# Autodesk Inventor assembly: Quadcopter Assembly
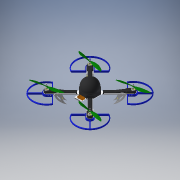
[picture p0: Inventor's stored thumbnail of the model, 180x180]
Saved by Autodesk Inventor 2016 (Build 200138000, 138)
## iProperties
Created: 2015-05-14
Part Number: Quadcopter Assembly
Document SubType Name: Assembly
Designer: Admin
Author: Admin
## Documents named in this file (16)
- E:\Documents\GITHUB\Side-Projects\Quadcopter\Quadcopter Assembly.iam
- E:\Documents\GITHUB\Side-Projects\Quadcopter\Arm.ipt
- E:\Documents\GITHUB\Side-Projects\Quadcopter\Body.ipt
- E:\Documents\GITHUB\Side-Projects\Quadcopter\ArmCover.ipt
- E:\Documents\GITHUB\Side-Projects\Quadcopter\MotorFull.ipt
- E:\Documents\GITHUB\Side-Projects\Quadcopter\Drone propeller guard.ipt
- E:\Documents\GITHUB\Side-Projects\Quadcopter\Motor top.ipt
- E:\Documents\GITHUB\Side-Projects\Quadcopter\propeller.ipt
- E:\Documents\GITHUB\Side-Projects\Quadcopter\Drone Cover.ipt
- E:\Documents\GITHUB\Side-Projects\Quadcopter\landing-gear-ublock.ipt
- E:\Documents\GITHUB\Side-Projects\Quadcopter\landing-gear-claws.ipt
- E:\Documents\GITHUB\Side-Projects\Quadcopter\clawholder.ipt
- E:\Documents\GITHUB\Side-Projects\Quadcopter\screw.ipt
- E:\Documents\GITHUB\Side-Projects\Quadcopter\control board.ipt
- E:\Documents\GITHUB\Side-Projects\Quadcopter\receiver.ipt
- E:\Documents\GITHUB\Side-Projects\Quadcopter\nut.ipt
## Components (112 placed, 15 different names)
1. Arm:1 — Mate:3, Rotational:2, Mate:8, Mate:32, Mate:35, Mate:52
2. Arm:2 — Mate:4, Rotational:4, Mate:10, Mate:17, Mate:18, Mate:28, Mate:29
3. Arm:3 — Mate:2, Rotational:3, Mate:5, Mate:13, Mate:14, Mate:49, Mate:50
4. Arm:4 — Mate:1, Rotational:1, Mate:12, Mate:43, Mate:44, Mate:45, Mate:46, Mate:47
5. Body:1 — Rotational:1, Rotational:2, Rotational:3, Rotational:4, Mate:25, Mate:26, Mate:27, Mate:51, Insert:5, Insert:6, Insert:7, Insert:8, Insert:9, Insert:10, Insert:11, Insert:12, Mate:53, Mate:54
6. ArmCover:1 — Mate:8
7. ArmCover:2 — Mate:5
8. ArmCover:3 — Mate:12
9. ArmCover:4 — Mate:10
10. MotorFull:1 — Mate:4, Mate:21
11. MotorFull:2 — Mate:3, Mate:24
12. MotorFull:3 — Mate:2, Mate:23
13. MotorFull:4 — Mate:1, Mate:22
14. Drone propeller guard:1 — Mate:13, Mate:14, Insert:49, Insert:50, Insert:59, Insert:60
15. Drone propeller guard:2 — Mate:52, Insert:55, Insert:56, Insert:61, Insert:62
16. Drone propeller guard:3 — Mate:17, Mate:18, Insert:53, Insert:54, Insert:63, Insert:64
17. Drone propeller guard:4 — Mate:43, Mate:44, Mate:45, Insert:51, Insert:52, Insert:57, Insert:58
18. Motor top:1 — Mate:24, Rotational:6, Insert:16, Insert:17, Insert:18
19. Motor top:2 — Mate:23, Rotational:8, Insert:13, Insert:14, Insert:15
20. Motor top:3 — Mate:22, Rotational:5, Insert:22, Insert:23, Insert:24
21. Motor top:4 — Mate:21, Rotational:7, Insert:19, Insert:20, Insert:21
22. propeller:1 — Rotational:5, Mate:58
23. propeller:2 — Rotational:6, Mate:55
24. propeller:3 — Rotational:7, Mate:57
25. propeller:4 — Rotational:8, Mate:56
26. Drone Cover:1 — Mate:25, Mate:26, Mate:27
27. landing-gear-ublock:2 — Mate:32, Mate:35, Rotational:9, Rotational:12
28. landing-gear-ublock:4 — Mate:28, Mate:29, Rotational:13, Rotational:15
29. landing-gear-claws:2 — Rotational:12, Mate:37, Insert:25, Insert:26, Insert:27
30. landing-gear-claws:3 — Rotational:13, Mate:41, Insert:31, Insert:32, Insert:48
31. landing-gear-claws:4 — Rotational:15, Mate:40, Insert:36, Insert:37, Insert:38
32. landing-gear-claws:5 — Mate:38, Rotational:17, Insert:28, Insert:29, Insert:30
33. landing-gear-claws:6 — Rotational:16, Mate:48, Insert:42, Insert:43, Insert:44
34. landing-gear-claws:7 — Rotational:9, Mate:36, Insert:39, Insert:40, Insert:41
35. clawholder:1
36. clawholder:2 — Mate:40, Mate:41
37. clawholder:3 — Mate:36, Mate:37
38. clawholder:4 — Mate:38, Mate:48
39. landing-gear-ublock:5 — Mate:46, Mate:47, Rotational:16, Rotational:17
40. landing-gear-ublock:6 — Mate:49, Mate:50, Rotational:18, Rotational:19
41. landing-gear-claws:8 — Rotational:18, Insert:45, Insert:46, Insert:47
42. landing-gear-claws:9 — Rotational:19, Insert:33, Insert:34, Insert:35
43. screw:1 — Insert:59
44. screw:2 — Insert:48
45. screw:3 — Insert:55
46. screw:4 — Insert:47
47. screw:5 — Insert:37
48. screw:6 — Insert:43
49. screw:7 — Insert:36
50. screw:8 — Insert:23
51. screw:9 — Insert:57
52. screw:10 — Insert:64
53. screw:11 — Insert:49
54. screw:12 — Insert:21
55. screw:13 — Insert:15
56. screw:14 — Insert:14
57. screw:15 — Insert:56
58. screw:19 — Insert:13
59. screw:20 — Insert:52
60. screw:21 — Insert:60
61. screw:22 — Insert:35
62. screw:23 — Insert:46
63. screw:24 — Insert:51
64. screw:25 — Insert:50
65. screw:26 — Insert:30
66. screw:27 — Insert:26
67. screw:28 — Insert:1
68. screw:29 — Insert:2
69. screw:30 — Insert:6
70. screw:31 — Insert:4
71. screw:32 — Insert:5
72. screw:33 — Insert:7
73. screw:34 — Insert:3
74. screw:35 — Insert:10
75. screw:36 — Insert:18
76. screw:37 — Insert:33
77. screw:38 — Insert:31
78. screw:39 — Insert:38
79. screw:40 — Insert:41
80. screw:41 — Insert:39
81. screw:43 — Insert:63
82. screw:44 — Insert:62
83. screw:45 — Insert:61
84. screw:46 — Insert:54
85. screw:47 — Insert:42
86. screw:48 — Insert:44
87. screw:49 — Insert:34
88. screw:50 — Insert:27
89. screw:51 — Insert:16
90. screw:52 — Insert:11
91. screw:53 — Insert:9
92. screw:54 — Insert:8
93. screw:55 — Insert:12
94. screw:56 — Insert:25
95. screw:57 — Insert:19
96. screw:58 — Insert:53
97. screw:59 — Insert:40
98. screw:60 — Insert:58
99. screw:61 — Insert:32
100. screw:62 — Insert:22
101. screw:63 — Insert:20
102. screw:64 — Insert:45
103. screw:65 — Insert:29
104. screw:66 — Insert:28
105. screw:67 — Insert:17
106. screw:68 — Insert:24
107. control board:1 — Mate:51, Insert:1, Insert:2, Insert:3, Insert:4
108. receiver:1 — Mate:53, Mate:54
109. nut:1 — Mate:57
110. nut:2 — Mate:55
111. nut:3 — Mate:58
112. nut:4 — Mate:56
## Relationships (124: Insert 64, Mate 44, RevoluteJoint 16)
- Mate:1: Arm:4 ↔ MotorFull:4
- Mate:2: Arm:3 ↔ MotorFull:3
- Mate:3: Arm:1 ↔ MotorFull:2
- Mate:4: Arm:2 ↔ MotorFull:1
- Rotational:1 [RevoluteJoint]: Arm:4 ↔ Body:1
- Rotational:2 [RevoluteJoint]: Arm:1 ↔ Body:1
- Rotational:3 [RevoluteJoint]: Arm:3 ↔ Body:1
- Rotational:4 [RevoluteJoint]: Arm:2 ↔ Body:1
- Mate:5: Arm:3 ↔ ArmCover:2
- Mate:8: Arm:1 ↔ ArmCover:1
- Mate:10: Arm:2 ↔ ArmCover:4
- Mate:12: Arm:4 ↔ ArmCover:3
- Mate:13: Arm:3 ↔ Drone propeller guard:1
- Mate:14: Arm:3 ↔ Drone propeller guard:1
- Mate:17: Arm:2 ↔ Drone propeller guard:3
- Mate:18: Arm:2 ↔ Drone propeller guard:3
- Mate:21: MotorFull:1 ↔ Motor top:4
- Mate:22: MotorFull:4 ↔ Motor top:3
- Mate:23: MotorFull:3 ↔ Motor top:2
- Mate:24: MotorFull:2 ↔ Motor top:1
- Rotational:5 [RevoluteJoint] (-4.5974 mm): Motor top:3 ↔ propeller:1
- Rotational:6 [RevoluteJoint] (-4.5974 mm): Motor top:1 ↔ propeller:2
- Rotational:7 [RevoluteJoint] (4.5974 mm): Motor top:4 ↔ propeller:3
- Rotational:8 [RevoluteJoint] (-4.5974 mm): Motor top:2 ↔ propeller:4
- Mate:25: Body:1 ↔ Drone Cover:1
- Mate:26: Body:1 ↔ Drone Cover:1
- Mate:27: Body:1 ↔ Drone Cover:1
- Mate:28: Arm:2 ↔ landing-gear-ublock:4
- Mate:29: Arm:2 ↔ landing-gear-ublock:4
- Mate:32: Arm:1 ↔ landing-gear-ublock:2
- Mate:35: Arm:1 ↔ landing-gear-ublock:2
- Rotational:9 [RevoluteJoint]: landing-gear-ublock:2 ↔ landing-gear-claws:7
- Rotational:12 [RevoluteJoint]: landing-gear-ublock:2 ↔ landing-gear-claws:2
- Rotational:13 [RevoluteJoint]: landing-gear-ublock:4 ↔ landing-gear-claws:3
- Rotational:15 [RevoluteJoint]: landing-gear-ublock:4 ↔ landing-gear-claws:4
- Mate:36: landing-gear-claws:7 ↔ clawholder:3
- Mate:37: landing-gear-claws:2 ↔ clawholder:3
- Mate:38: landing-gear-claws:5 ↔ clawholder:4
- Mate:40: landing-gear-claws:4 ↔ clawholder:2
- Mate:41: landing-gear-claws:3 ↔ clawholder:2
- Mate:43: Arm:4 ↔ Drone propeller guard:4
- Mate:44: Arm:4 ↔ Drone propeller guard:4
- Mate:45: Arm:4 ↔ Drone propeller guard:4
- Mate:46: Arm:4 ↔ landing-gear-ublock:5
- Mate:47: Arm:4 ↔ landing-gear-ublock:5
- Rotational:16 [RevoluteJoint]: landing-gear-claws:6 ↔ landing-gear-ublock:5
- Rotational:17 [RevoluteJoint]: landing-gear-claws:5 ↔ landing-gear-ublock:5
- Mate:48: landing-gear-claws:6 ↔ clawholder:4
- Mate:49: Arm:3 ↔ landing-gear-ublock:6
- Mate:50: Arm:3 ↔ landing-gear-ublock:6
- Rotational:18 [RevoluteJoint]: landing-gear-ublock:6 ↔ landing-gear-claws:8
- Rotational:19 [RevoluteJoint]: landing-gear-ublock:6 ↔ landing-gear-claws:9
- Mate:51: Body:1 ↔ control board:1
- Insert:1 (-12.4968 mm): screw:28 ↔ control board:1
- Insert:2 (-12.4968 mm): screw:29 ↔ control board:1
- Insert:3 (-12.4968 mm): screw:34 ↔ control board:1
- Insert:4 (-12.4968 mm): screw:31 ↔ control board:1
- Insert:5 (-12.4968 mm): Body:1 ↔ screw:32
- Insert:6 (-12.4968 mm): Body:1 ↔ screw:30
- Insert:7 (-12.4968 mm): Body:1 ↔ screw:33
- Insert:8 (-12.4968 mm): Body:1 ↔ screw:54
- Insert:9 (-12.4968 mm): Body:1 ↔ screw:53
- Insert:10 (-12.4968 mm): Body:1 ↔ screw:35
- Insert:11 (-12.4968 mm): Body:1 ↔ screw:52
- Insert:12 (-12.4968 mm): Body:1 ↔ screw:55
- Insert:13 (-12.4968 mm): Motor top:2 ↔ screw:19
- Insert:14 (-12.4968 mm): Motor top:2 ↔ screw:14
- Insert:15 (-12.4968 mm): Motor top:2 ↔ screw:13
- Insert:16 (-12.4968 mm): Motor top:1 ↔ screw:51
- Insert:17 (-12.4968 mm): Motor top:1 ↔ screw:67
- Insert:18 (-12.4968 mm): Motor top:1 ↔ screw:36
- Insert:19 (-12.4968 mm): Motor top:4 ↔ screw:57
- Insert:20 (-12.4968 mm): Motor top:4 ↔ screw:63
- Insert:21 (-12.4968 mm): Motor top:4 ↔ screw:12
- Insert:22 (-12.4968 mm): Motor top:3 ↔ screw:62
- Insert:23 (-12.4968 mm): Motor top:3 ↔ screw:8
- Insert:24 (-12.4968 mm): Motor top:3 ↔ screw:68
- Insert:25 (-12.4968 mm): landing-gear-claws:2 ↔ screw:56
- Insert:26 (-12.4968 mm): landing-gear-claws:2 ↔ screw:27
- Insert:27 (-12.4968 mm): landing-gear-claws:2 ↔ screw:50
- Insert:28 (-12.4968 mm): landing-gear-claws:5 ↔ screw:66
- Insert:29 (-12.4968 mm): landing-gear-claws:5 ↔ screw:65
- Insert:30 (-12.4968 mm): landing-gear-claws:5 ↔ screw:26
- Insert:31 (-12.4968 mm): landing-gear-claws:3 ↔ screw:38
- Insert:32 (-12.4968 mm): landing-gear-claws:3 ↔ screw:61
- Insert:33 (-12.4968 mm): landing-gear-claws:9 ↔ screw:37
- Insert:34 (-12.4968 mm): landing-gear-claws:9 ↔ screw:49
- Insert:35 (-12.4968 mm): landing-gear-claws:9 ↔ screw:22
- Insert:36 (-12.4968 mm): landing-gear-claws:4 ↔ screw:7
- Insert:37 (-12.4968 mm): landing-gear-claws:4 ↔ screw:5
- Insert:38 (-12.4968 mm): landing-gear-claws:4 ↔ screw:39
- Insert:39 (-12.4968 mm): landing-gear-claws:7 ↔ screw:41
- Insert:40 (-12.4968 mm): landing-gear-claws:7 ↔ screw:59
- Insert:41 (-12.4968 mm): landing-gear-claws:7 ↔ screw:40
- Insert:42 (-12.4968 mm): landing-gear-claws:6 ↔ screw:47
- Insert:43 (-12.4968 mm): landing-gear-claws:6 ↔ screw:6
- Insert:44 (-12.4968 mm): landing-gear-claws:6 ↔ screw:48
- Insert:45 (-12.4968 mm): landing-gear-claws:8 ↔ screw:64
- Insert:46 (-12.4968 mm): landing-gear-claws:8 ↔ screw:23
- Insert:47 (-12.4968 mm): landing-gear-claws:8 ↔ screw:4
- Insert:48 (-12.4968 mm): landing-gear-claws:3 ↔ screw:2
- Insert:49 (-12.4968 mm): Drone propeller guard:1 ↔ screw:11
- Insert:50 (-12.4968 mm): Drone propeller guard:1 ↔ screw:25
- Insert:51 (-12.4968 mm): Drone propeller guard:4 ↔ screw:24
- Insert:52 (-12.4968 mm): Drone propeller guard:4 ↔ screw:20
- Insert:53 (-12.4968 mm): Drone propeller guard:3 ↔ screw:58
- Insert:54 (-12.4968 mm): Drone propeller guard:3 ↔ screw:46
- Mate:52: Arm:1 ↔ Drone propeller guard:2
- Insert:55 (-12.4968 mm): Drone propeller guard:2 ↔ screw:3
- Insert:56 (-12.4968 mm): Drone propeller guard:2 ↔ screw:15
- Insert:57 (-12.4968 mm): Drone propeller guard:4 ↔ screw:9
- Insert:58 (-12.4968 mm): Drone propeller guard:4 ↔ screw:60
- Insert:59 (-12.4968 mm): Drone propeller guard:1 ↔ screw:1
- Insert:60 (-12.4968 mm): Drone propeller guard:1 ↔ screw:21
- Insert:61 (-12.4968 mm): Drone propeller guard:2 ↔ screw:45
- Insert:62 (-12.4968 mm): Drone propeller guard:2 ↔ screw:44
- Insert:63 (-12.4968 mm): Drone propeller guard:3 ↔ screw:43
- Insert:64 (-12.4968 mm): Drone propeller guard:3 ↔ screw:10
- Mate:53: Body:1 ↔ receiver:1
- Mate:54: Body:1 ↔ receiver:1
- Mate:55: propeller:2 ↔ nut:2
- Mate:56: propeller:4 ↔ nut:4
- Mate:57: propeller:3 ↔ nut:1
- Mate:58: propeller:1 ↔ nut:3
